# Autodesk Inventor assembly: LinearLift12in
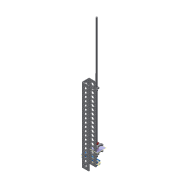
[picture p0: Inventor's stored thumbnail of the model, 180x180]
Saved by Autodesk Inventor 2018 (Build 220112000, 112)
## iProperties
Created: 2017-11-27
Part Number: LinearLift12in
Document SubType Name: Assembly
Designer: ball
Author: ball
## Documents named in this file (6)
- C:\FTC\FTC8863CAD\2017Robot\LinearLift12in.iam
- C:\FTC\FTC8863CAD\Actobotics\585 parts\585634.ipt
- C:\FTC\FTC8863CAD\Actobotics\585 parts\585458.ipt
- C:\FTC\FTC8863CAD\2017Robot\LinearBearingPlusClamps.iam
- C:\FTC\FTC8863CAD\Actobotics\634 parts\634315.ipt
- C:\FTC\FTC8863CAD\Actobotics\565 parts\565018.ipt
## Components (6 placed, 5 different names)
1. 585458:2 — Mate:44, Angle:1, Mate:49, Mate:50, Mate:51, Mate:52, Mate:53, Flush:6, Mate:54, Mate:55
2. 585634:5 — Mate:44, Flush:5, Mate:47, Mate:48, Mate:54, Mate:55
3. 634315:1 — Flush:5, Mate:46, Mate:48
4. LinearBearingPlusClamps:2 [sub-assembly] — Mate:46, Angle:1, Mate:47
5. 585634:7 — Mate:49, Mate:50, Mate:51
6. 565018:1 — Mate:52, Mate:53, Flush:6
## Relationships (14: Mate 11, Flush 2, Angle 1)
- Mate:44: 585458:2 ↔ 585634:5
- Flush:5: 585634:5 ↔ 634315:1
- Mate:46: 634315:1 ↔ LinearBearingPlusClamps:2
- Angle:1 (0 deg): 585458:2 ↔ LinearBearingPlusClamps:2
- Mate:47: 585634:5 ↔ LinearBearingPlusClamps:2
- Mate:48: 585634:5 ↔ 634315:1
- Mate:49: 585458:2 ↔ 585634:7
- Mate:50: 585458:2 ↔ 585634:7
- Mate:51: 585458:2 ↔ 585634:7
- Mate:52: 585458:2 ↔ 565018:1
- Mate:53: 585458:2 ↔ 565018:1
- Flush:6: 585458:2 ↔ 565018:1
- Mate:54: 585458:2 ↔ 585634:5
- Mate:55: 585458:2 ↔ 585634:5
